# Autodesk Inventor assembly: MX-106T+idle.ipt
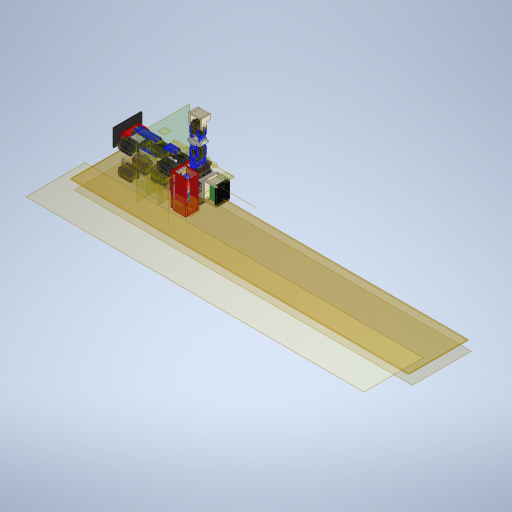
[picture p0: Inventor's stored thumbnail of the model, 512x512]
Saved by Autodesk Inventor 2024 (Build 280153000, 153)
## iProperties
Created: 2022-08-09
Part Number: MX-106T+idle.ipt
Document SubType Name: Assembly
Designer: 박지훈
Author: 박지훈
## Documents named in this file (48)
- C:\Users\Eungang\Documents\Inventor\Fighting_Robot\다이나믹셀\MX-106T+idle.ipt.iam
- C:\Users\Eungang\Documents\Inventor\Fighting_Robot\아이들러\64아이들러.iam
- C:\Users\Eungang\Documents\Inventor\Fighting_Robot\다이나믹셀\MX-106T.ipt
- C:\Users\Eungang\Documents\Inventor\Fighting_Robot\혼\64-106Horn.ipt
- C:\Users\Eungang\Documents\Inventor\Fighting_Robot\new_foot_connect.ipt
- C:\Users\Eungang\Documents\Inventor\Fighting_Robot\foot_2.ipt
- C:\Users\Eungang\Documents\Inventor\Fighting_Robot\new_foot_connect_1.ipt
- C:\Users\Eungang\Documents\Inventor\Fighting_Robot\다이나믹셀\MX-64T.ipt
- C:\Users\Eungang\Documents\Inventor\Fighting_Robot\new_waist.ipt
- C:\Users\Eungang\Documents\Inventor\Fighting_Robot\foot_connect_3_MIR1_MIR1.ipt
- C:\Users\Eungang\Documents\Inventor\Fighting_Robot\real_waist.ipt
- C:\Users\Eungang\Documents\Inventor\Fighting_Robot\Enrichpower_2200mAh_11.1V_30C.ipt
- C:\Users\Eungang\Documents\Inventor\Fighting_Robot\다이나믹셀\MX-28T_R.ipt
- C:\Users\Eungang\Documents\Inventor\Fighting_Robot\혼\28Horn.ipt
- C:\Users\Eungang\Documents\Inventor\Fighting_Robot\아이들러\28아이들러.iam
- C:\Users\Eungang\Documents\Inventor\Fighting_Robot\arm_connect_3.ipt
- C:\Users\Eungang\Documents\Inventor\Fighting_Robot\arm_connect_5.ipt
- C:\Users\Eungang\Documents\Inventor\Fighting_Robot\arm_connect_7.ipt
- C:\Users\Eungang\Documents\Inventor\Fighting_Robot\MOLRA.ipt
- C:\Users\Eungang\Documents\Inventor\Fighting_Robot\a.ipt
- C:\Users\Eungang\Documents\Inventor\Fighting_Robot\Circuit.ipt
- C:\Users\Eungang\Documents\Inventor\Fighting_Robot\neck.ipt
- C:\Users\Eungang\Documents\Inventor\Fighting_Robot\b.ipt
- C:\Users\Eungang\Documents\Inventor\Fighting_Robot\arm_connect_5_MIR.ipt
- C:\Users\Eungang\Documents\Inventor\Fighting_Robot\c.ipt
- C:\Users\Eungang\Documents\Inventor\Fighting_Robot\D.ipt
- C:\Users\Eungang\Documents\Inventor\Fighting_Robot\E.ipt
- C:\Users\Eungang\Documents\Inventor\Fighting_Robot\afdas.ipt
- C:\Users\Eungang\Documents\Inventor\Fighting_Robot\afsd.ipt
- C:\Users\Eungang\Documents\Inventor\Fighting_Robot\afsd_MIR.ipt
- C:\Users\Eungang\Documents\Inventor\Fighting_Robot\adsa.ipt
- C:\Users\Eungang\Documents\Inventor\Fighting_Robot\부품43.ipt
- C:\Users\Eungang\Documents\Inventor\Fighting_Robot\부품44.ipt
- C:\Users\Eungang\Documents\Inventor\Fighting_Robot\64horn.ipt
- C:\Users\Eungang\Documents\Inventor\Fighting_Robot\부품46.ipt
- C:\Users\Eungang\Documents\Inventor\Fighting_Robot\부품47.ipt
- C:\Users\Eungang\Documents\Inventor\Fighting_Robot\부품48.ipt
- C:\Users\Eungang\Documents\Inventor\Fighting_Robot\부품49.ipt
- C:\Users\Eungang\Documents\Inventor\Fighting_Robot\부품50.ipt
- C:\Users\Eungang\Documents\Inventor\Fighting_Robot\부품51.ipt
- C:\Users\Eungang\Documents\Inventor\Fighting_Robot\부품52.ipt
- C:\Users\Eungang\Documents\Inventor\Fighting_Robot\부품53.ipt
- C:\Users\Eungang\Documents\Inventor\Fighting_Robot\부품54.ipt
- C:\Users\Eungang\Documents\Inventor\Fighting_Robot\부품56.ipt
- C:\Users\Eungang\Documents\Inventor\Fighting_Robot\final.ipt
- C:\Users\Eungang\Documents\Inventor\Fighting_Robot\sad.ipt
- C:\Users\Eungang\Documents\Inventor\Fighting_Robot\부품48_MIR.ipt
- C:\Users\Eungang\Documents\Inventor\Fighting_Robot\foot_connect_3_MIR1_MIR1_MIR.ipt
## Components (99 placed, 47 different names)
1. 64-106Horn:1 — 메이트:11, 삽입:35
2. 64-106Horn:2 — 삽입:157, 메이트:405
3. new_foot_connect:2 — 메이트:11, 삽입:180
4. foot_2:1 — 삽입:180, 메이트:402, 플러쉬:100
5. 64-106Horn:5 — 삽입:150, 메이트:404
6. 64아이들러:2 [sub-assembly] — 삽입:165
7. 64아이들러:5 [sub-assembly] — 삽입:164
8. new_foot_connect_1:2
9. MX-64T:3 — 삽입:35, 메이트:325, 플러쉬:77
10. 64아이들러:6 [sub-assembly] — 삽입:189, 플러쉬:88, 메이트:347
11. real_waist:2 — 메이트:218, 플러쉬:78, 메이트:382, 메이트:385, 메이트:396
12. MX-64T:10 — 삽입:100, 삽입:116, 메이트:207, 플러쉬:65, 메이트:360
13. 64-106Horn:12 — 삽입:100, 삽입:185, 삽입:186
14. 64-106Horn:14 — 삽입:117, 메이트:219, 삽입:138
15. arm_connect_7:1
16. a:1 — 메이트:250, 플러쉬:67, 메이트:372, 메이트:374, 메이트:375, 메이트:376
17. 64아이들러:11 [sub-assembly] — 삽입:116
18. neck:1
19. Circuit:1 — 메이트:250, 메이트:370, 메이트:373
20. arm_connect_5:5
21. MX-64T:11 — 플러쉬:65, 메이트:218, 삽입:117, 메이트:219, 플러쉬:66, 메이트:241, 메이트:242, 메이트:337, 플러쉬:79, 메이트:361, 삽입:198, 삽입:199
22. arm_connect_5:6
23. arm_connect_5:7 — 메이트:380, 메이트:381
24. b:1 — 플러쉬:66
25. arm_connect_5:8 — 메이트:377, 메이트:378
26. arm_connect_5_MIR:1
27. MX-28T_R:4 — 메이트:241, 메이트:242, 플러쉬:68, 삽입:132, 삽입:135, 메이트:259
28. c:1 — 플러쉬:67, 메이트:353, 메이트:354, 메이트:355, 메이트:370, 메이트:372, 메이트:373, 메이트:374
29. a:3 — 메이트:353, 메이트:354, 메이트:355
30. D:1 — 플러쉬:68
31. 28Horn:5 — 삽입:132, 삽입:133, 메이트:259
32. arm_connect_3:1 — 삽입:133, 메이트:258
33. 28아이들러:1 [sub-assembly] — 삽입:135, 삽입:136, 삽입:137
34. arm_connect_3:2 — 삽입:136, 삽입:137, 플러쉬:69, 메이트:257
35. E:1 — 플러쉬:69, 메이트:257, 메이트:258, 삽입:138
36. MX-106T:8 — 삽입:150, 삽입:164, 플러쉬:75, 삽입:176, 플러쉬:85, 플러쉬:86, 메이트:345, 삽입:182, 삽입:183, 삽입:184, 메이트:404, 플러쉬:104
37. new_foot_connect_1:3
38. MX-28T_R:5 — 삽입:159, 메이트:289, 메이트:290, 메이트:291, 삽입:201, 메이트:397
39. MX-106T:9 — 삽입:157, 삽입:165, 플러쉬:75, 메이트:325, 플러쉬:77, 메이트:405, 플러쉬:101, 플러쉬:103, 메이트:406, 메이트:407, 메이트:408, 메이트:409
40. 28Horn:6 — 삽입:159, 메이트:289, 메이트:290, 메이트:291, 플러쉬:93, 삽입:200
41. afdas:1
42. foot_connect_3_MIR1_MIR1:2 — 삽입:177
43. afsd_MIR:1 — 삽입:176, 삽입:182
44. new_waist:1 — 삽입:178, 삽입:179, 플러쉬:91, 플러쉬:92, 메이트:356, 메이트:357, 메이트:358, 대칭:2
45. 64아이들러:12 [sub-assembly] — 삽입:177, 삽입:178, 삽입:179
46. adsa:1 — 플러쉬:79
47. 부품43:1
48. MX-106T:10 — 플러쉬:85, 플러쉬:86, 메이트:344, 메이트:345, 삽입:189, 메이트:347, 삽입:190, 플러쉬:89, 메이트:352, 플러쉬:90, 메이트:361, 플러쉬:108
49. 부품44:1
50. afsd:1 — 삽입:183, 삽입:184
51. 64horn:2 — 삽입:185, 삽입:186, 메이트:359
52. 부품47:1 — 플러쉬:88
53. 64-106Horn:17 — 삽입:190, 삽입:191, 삽입:192
54. 부품46:1 — 삽입:191, 삽입:192
55. 64-106Horn:18 — 삽입:194
56. MX-64T:12 — 삽입:194, 플러쉬:89, 메이트:352
57. 부품48:1 — 플러쉬:90
58. 부품49:1 — 메이트:356, 메이트:357, 메이트:358, 메이트:359, 대칭:2
59. MX-64T:14 — 플러쉬:102, 플러쉬:105
60. 부품51:1 — 삽입:198, 삽입:199, 메이트:375, 메이트:376
61. 부품52:1 — 메이트:377, 메이트:378, 메이트:380, 메이트:381
62. 부품50:1 — 메이트:382, 메이트:386, 메이트:387
63. MOLRA:6 — 메이트:391, 메이트:392, 메이트:393
64. 부품50:2 — 메이트:388, 메이트:389, 메이트:390, 메이트:391, 메이트:392, 메이트:393
65. MOLRA:7 — 메이트:385, 메이트:386, 메이트:387, 메이트:388, 메이트:389, 메이트:390
66. Enrichpower_2200mAh_11.1V_30C:1 — 메이트:396
67. 부품53:1 — 플러쉬:93, 삽입:200, 메이트:401
68. 28아이들러:2 [sub-assembly] — 삽입:201, 메이트:397, 플러쉬:95, 삽입:202
69. 부품56:1 — 플러쉬:95, 메이트:398, 메이트:399, 메이트:400, 삽입:202
70. 부품54:1 — 메이트:398, 메이트:399, 메이트:400, 메이트:401
71. final:1 — 메이트:402, 플러쉬:100
72. sad:1 — 플러쉬:101
73. MX-106T:11 — 플러쉬:102, 플러쉬:103, 메이트:406, 플러쉬:106, 삽입:208, 메이트:410, 삽입:212, 삽입:225, 메이트:412, 플러쉬:110, 플러쉬:111, 메이트:415
74. MX-106T:12 — 플러쉬:104, 플러쉬:105, 플러쉬:106, 플러쉬:107, 플러쉬:109, 삽입:205, 삽입:209, 삽입:216, 삽입:217, 삽입:219, 삽입:220
75. new_foot_connect:3 — 삽입:204
76. 64아이들러:13 [sub-assembly] — 삽입:203, 삽입:204
77. 부품48_MIR:1 — 메이트:407, 메이트:408, 메이트:409, 삽입:203
78. MX-106T:13 — 플러쉬:107, 플러쉬:108, 플러쉬:109, 삽입:207, 삽입:210, 삽입:222, 삽입:223
79. 64아이들러:14 [sub-assembly] — 삽입:205, 삽입:214
80. 64아이들러:16 [sub-assembly] — 삽입:207, 삽입:215
81. 64-106Horn:19 — 삽입:208
82. 64-106Horn:20 — 삽입:210, 삽입:221
83. 64-106Horn:21 — 삽입:209, 삽입:211
84. new_foot_connect_1:4 — 삽입:211, 메이트:410
85. new_foot_connect_1:5 — 삽입:213, 삽입:214
86. 64아이들러:17 [sub-assembly] — 삽입:212, 삽입:213
87. 부품47:3 — 삽입:215, 삽입:218
88. afsd_MIR:2 — 삽입:216, 삽입:217, 삽입:218
89. 부품46:2 — 삽입:221, 메이트:411
90. afsd:2 — 삽입:219, 삽입:220, 메이트:411
91. foot_connect_3_MIR1_MIR1_MIR:1 — 삽입:222, 삽입:223, 삽입:224
92. 64아이들러:18 [sub-assembly] — 삽입:224
93. 부품48_MIR:2 — 삽입:225, 메이트:412, 삽입:226
94. new_foot_connect:4 — 삽입:227, 삽입:228, 메이트:413, 메이트:415
95. 64아이들러:19 [sub-assembly] — 삽입:226, 삽입:227
96. foot_2:2 — 삽입:228, 메이트:413, 삽입:229, 삽입:230
97. new_foot_connect:5 — 삽입:229, 삽입:230, 메이트:414
98. MX-64T:15 — 플러쉬:110, 플러쉬:111
99. 64-106Horn:22 — 메이트:414
## Relationships (163: Mate 68, Insert 62, Flush 32, Symmetry 1)
- 플러쉬:1 [Flush] (-30 mm)
- 플러쉬:2 [Flush] (30 mm)
- 메이트:11 [Mate]: 64-106Horn:1 ↔ new_foot_connect:2
- 삽입:35 [Insert] (0.5 mm): 64-106Horn:1 ↔ MX-64T:3
- 삽입:100 [Insert] (0.5 mm): MX-64T:10 ↔ 64-106Horn:12
- 삽입:116 [Insert] (0.5 mm): MX-64T:10 ↔ 64아이들러:11
- 메이트:207 [Mate]: MX-64T:10
- 플러쉬:65 [Flush]: MX-64T:10 ↔ MX-64T:11
- 메이트:218 [Mate]: real_waist:2 ↔ MX-64T:11
- 삽입:117 [Insert] (0.5 mm): 64-106Horn:14 ↔ MX-64T:11
- 메이트:219 [Mate]: 64-106Horn:14 ↔ MX-64T:11
- 플러쉬:66 [Flush]: MX-64T:11 ↔ b:1
- 메이트:241 [Mate]: MX-64T:11 ↔ MX-28T_R:4
- 메이트:242 [Mate]: MX-64T:11 ↔ MX-28T_R:4
- 메이트:250 [Mate] (10 mm): a:1 ↔ Circuit:1
- 플러쉬:67 [Flush]: a:1 ↔ c:1
- 플러쉬:68 [Flush]: MX-28T_R:4 ↔ D:1
- 삽입:132 [Insert] (0.75 mm): MX-28T_R:4 ↔ 28Horn:5
- 삽입:133 [Insert]: 28Horn:5 ↔ arm_connect_3:1
- 삽입:135 [Insert] (0.75 mm): MX-28T_R:4 ↔ 28아이들러:1
- 삽입:136 [Insert]: 28아이들러:1 ↔ arm_connect_3:2
- 삽입:137 [Insert]: 28아이들러:1 ↔ arm_connect_3:2
- 플러쉬:69 [Flush]: arm_connect_3:2 ↔ E:1
- 메이트:257 [Mate]: arm_connect_3:2 ↔ E:1
- 메이트:258 [Mate]: arm_connect_3:1 ↔ E:1
- 메이트:259 [Mate]: MX-28T_R:4 ↔ 28Horn:5
- 삽입:138 [Insert] (0.1 mm): 64-106Horn:14 ↔ E:1
- 삽입:150 [Insert] (0.5 mm): 64-106Horn:5 ↔ MX-106T:8
- 삽입:157 [Insert] (0.5 mm): 64-106Horn:2 ↔ MX-106T:9
- 삽입:159 [Insert] (0.75 mm): MX-28T_R:5 ↔ 28Horn:6
- 메이트:289 [Mate]: MX-28T_R:5 ↔ 28Horn:6
- 메이트:290 [Mate]: MX-28T_R:5 ↔ 28Horn:6
- 메이트:291 [Mate]: MX-28T_R:5 ↔ 28Horn:6
- 삽입:164 [Insert] (0.5 mm): 64아이들러:5 ↔ MX-106T:8
- 삽입:165 [Insert] (0.5 mm): 64아이들러:2 ↔ MX-106T:9
- 플러쉬:75 [Flush]: MX-106T:8 ↔ MX-106T:9
- 삽입:176 [Insert]: MX-106T:8 ↔ afsd_MIR:1
- 메이트:324 [Mate]
- 메이트:325 [Mate]: MX-64T:3 ↔ MX-106T:9
- 플러쉬:77 [Flush]: MX-64T:3 ↔ MX-106T:9
- 삽입:177 [Insert] (0.1 mm): foot_connect_3_MIR1_MIR1:2 ↔ 64아이들러:12
- 삽입:178 [Insert]: new_waist:1 ↔ 64아이들러:12
- 삽입:179 [Insert]: new_waist:1 ↔ 64아이들러:12
- 플러쉬:78 [Flush] (-6 mm): real_waist:2
- 메이트:337 [Mate]: MX-64T:11
- 플러쉬:79 [Flush]: MX-64T:11 ↔ adsa:1
- 삽입:180 [Insert]: new_foot_connect:2 ↔ foot_2:1
- 플러쉬:85 [Flush]: MX-106T:8 ↔ MX-106T:10
- 플러쉬:86 [Flush]: MX-106T:8 ↔ MX-106T:10
- 메이트:344 [Mate]: MX-106T:10
- 메이트:345 [Mate] (20 mm): MX-106T:8 ↔ MX-106T:10
- 삽입:182 [Insert]: MX-106T:8 ↔ afsd_MIR:1
- 삽입:183 [Insert]: MX-106T:8 ↔ afsd:1
- 삽입:184 [Insert]: MX-106T:8 ↔ afsd:1
- 삽입:185 [Insert]: 64-106Horn:12 ↔ 64horn:2
- 삽입:186 [Insert]: 64-106Horn:12 ↔ 64horn:2
- 삽입:189 [Insert] (0.5 mm): 64아이들러:6 ↔ MX-106T:10
- 플러쉬:88 [Flush]: 64아이들러:6 ↔ 부품47:1
- 메이트:347 [Mate]: 64아이들러:6 ↔ MX-106T:10
- 삽입:190 [Insert] (0.5 mm): MX-106T:10 ↔ 64-106Horn:17
- 삽입:191 [Insert]: 64-106Horn:17 ↔ 부품46:1
- 삽입:192 [Insert]: 64-106Horn:17 ↔ 부품46:1
- 삽입:194 [Insert] (0.5 mm): 64-106Horn:18 ↔ MX-64T:12
- 플러쉬:89 [Flush]: MX-106T:10 ↔ MX-64T:12
- 메이트:352 [Mate]: MX-106T:10 ↔ MX-64T:12
- 플러쉬:90 [Flush]: MX-106T:10 ↔ 부품48:1
- 메이트:353 [Mate]: c:1 ↔ a:3
- 메이트:354 [Mate]: c:1 ↔ a:3
- 메이트:355 [Mate]: c:1 ↔ a:3
- 플러쉬:91 [Flush]: new_waist:1
- 플러쉬:92 [Flush]: new_waist:1
- 메이트:356 [Mate]: new_waist:1 ↔ 부품49:1
- 메이트:357 [Mate]: new_waist:1 ↔ 부품49:1
- 메이트:358 [Mate]: new_waist:1 ↔ 부품49:1
- 메이트:359 [Mate]: 64horn:2 ↔ 부품49:1
- 대칭:2 [Symmetry]: new_waist:1 ↔ 부품49:1
- 메이트:360 [Mate]: MX-64T:10
- 메이트:361 [Mate]: MX-64T:11 ↔ MX-106T:10
- 메이트:370 [Mate] (0.2 mm): Circuit:1 ↔ c:1
- 메이트:372 [Mate]: a:1 ↔ c:1
- 메이트:373 [Mate] (0.2 mm): Circuit:1 ↔ c:1
- 삽입:198 [Insert]: MX-64T:11 ↔ 부품51:1
- 삽입:199 [Insert]: MX-64T:11 ↔ 부품51:1
- 메이트:374 [Mate]: a:1 ↔ c:1
- 메이트:375 [Mate]: a:1 ↔ 부품51:1
- 메이트:376 [Mate]: a:1 ↔ 부품51:1
- 메이트:377 [Mate] (0.1 mm): arm_connect_5:8 ↔ 부품52:1
- 메이트:378 [Mate]: arm_connect_5:8 ↔ 부품52:1
- 메이트:380 [Mate]: arm_connect_5:7 ↔ 부품52:1
- 메이트:381 [Mate]: arm_connect_5:7 ↔ 부품52:1
- 메이트:382 [Mate]: real_waist:2 ↔ 부품50:1
- 메이트:385 [Mate]: real_waist:2 ↔ MOLRA:7
- 메이트:386 [Mate]: 부품50:1 ↔ MOLRA:7
- 메이트:387 [Mate]: 부품50:1 ↔ MOLRA:7
- 메이트:388 [Mate]: 부품50:2 ↔ MOLRA:7
- 메이트:389 [Mate]: 부품50:2 ↔ MOLRA:7
- 메이트:390 [Mate]: 부품50:2 ↔ MOLRA:7
- 메이트:391 [Mate]: MOLRA:6 ↔ 부품50:2
- 메이트:392 [Mate]: MOLRA:6 ↔ 부품50:2
- 메이트:393 [Mate]: MOLRA:6 ↔ 부품50:2
- 메이트:396 [Mate]: real_waist:2 ↔ Enrichpower_2200mAh_11.1V_30C:1
- 플러쉬:93 [Flush]: 28Horn:6 ↔ 부품53:1
- 삽입:200 [Insert]: 28Horn:6 ↔ 부품53:1
- 삽입:201 [Insert] (0.5 mm): MX-28T_R:5 ↔ 28아이들러:2
- 메이트:397 [Mate]: MX-28T_R:5 ↔ 28아이들러:2
- 플러쉬:95 [Flush]: 28아이들러:2 ↔ 부품56:1
- 메이트:398 [Mate]: 부품56:1 ↔ 부품54:1
- 메이트:399 [Mate]: 부품56:1 ↔ 부품54:1
- 메이트:400 [Mate]: 부품56:1 ↔ 부품54:1
- 메이트:401 [Mate]: 부품53:1 ↔ 부품54:1
- 메이트:402 [Mate]: foot_2:1 ↔ final:1
- 플러쉬:100 [Flush] (-33 mm): foot_2:1 ↔ final:1
- 메이트:404 [Mate]: 64-106Horn:5 ↔ MX-106T:8
- 메이트:405 [Mate]: 64-106Horn:2 ↔ MX-106T:9
- 삽입:202 [Insert]: 28아이들러:2 ↔ 부품56:1
- 플러쉬:101 [Flush]: MX-106T:9 ↔ sad:1
- 플러쉬:102 [Flush]: MX-64T:14 ↔ MX-106T:11
- 플러쉬:103 [Flush]: MX-106T:9 ↔ MX-106T:11
- 메이트:406 [Mate]: MX-106T:9 ↔ MX-106T:11
- 플러쉬:104 [Flush]: MX-106T:8 ↔ MX-106T:12
- 플러쉬:105 [Flush]: MX-64T:14 ↔ MX-106T:12
- 플러쉬:106 [Flush]: MX-106T:11 ↔ MX-106T:12
- 메이트:407 [Mate]: MX-106T:9 ↔ 부품48_MIR:1
- 메이트:408 [Mate]: MX-106T:9 ↔ 부품48_MIR:1
- 메이트:409 [Mate]: MX-106T:9 ↔ 부품48_MIR:1
- 삽입:203 [Insert]: 64아이들러:13 ↔ 부품48_MIR:1
- 삽입:204 [Insert]: new_foot_connect:3 ↔ 64아이들러:13
- 플러쉬:107 [Flush]: MX-106T:12 ↔ MX-106T:13
- 플러쉬:108 [Flush]: MX-106T:10 ↔ MX-106T:13
- 플러쉬:109 [Flush]: MX-106T:12 ↔ MX-106T:13
- 삽입:205 [Insert] (0.5 mm): MX-106T:12 ↔ 64아이들러:14
- 삽입:207 [Insert] (0.5 mm): MX-106T:13 ↔ 64아이들러:16
- 삽입:208 [Insert] (0.5 mm): MX-106T:11 ↔ 64-106Horn:19
- 삽입:209 [Insert] (0.5 mm): MX-106T:12 ↔ 64-106Horn:21
- 삽입:210 [Insert] (0.5 mm): MX-106T:13 ↔ 64-106Horn:20
- 삽입:211 [Insert]: 64-106Horn:21 ↔ new_foot_connect_1:4
- 메이트:410 [Mate]: MX-106T:11 ↔ new_foot_connect_1:4
- 삽입:212 [Insert] (0.5 mm): MX-106T:11 ↔ 64아이들러:17
- 삽입:213 [Insert]: new_foot_connect_1:5 ↔ 64아이들러:17
- 삽입:214 [Insert]: 64아이들러:14 ↔ new_foot_connect_1:5
- 삽입:215 [Insert]: 64아이들러:16 ↔ 부품47:3
- 삽입:216 [Insert]: MX-106T:12 ↔ afsd_MIR:2
- 삽입:217 [Insert]: MX-106T:12 ↔ afsd_MIR:2
- 삽입:218 [Insert] (0.2 mm): 부품47:3 ↔ afsd_MIR:2
- 삽입:219 [Insert]: MX-106T:12 ↔ afsd:2
- 삽입:220 [Insert]: MX-106T:12 ↔ afsd:2
- 삽입:221 [Insert]: 64-106Horn:20 ↔ 부품46:2
- 메이트:411 [Mate] (0.2 mm): 부품46:2 ↔ afsd:2
- 삽입:222 [Insert]: MX-106T:13 ↔ foot_connect_3_MIR1_MIR1_MIR:1
- 삽입:223 [Insert]: MX-106T:13 ↔ foot_connect_3_MIR1_MIR1_MIR:1
- 삽입:224 [Insert]: foot_connect_3_MIR1_MIR1_MIR:1 ↔ 64아이들러:18
- 삽입:225 [Insert]: MX-106T:11 ↔ 부품48_MIR:2
- 메이트:412 [Mate]: MX-106T:11 ↔ 부품48_MIR:2
- 삽입:226 [Insert]: 부품48_MIR:2 ↔ 64아이들러:19
- 삽입:227 [Insert]: new_foot_connect:4 ↔ 64아이들러:19
- 삽입:228 [Insert]: new_foot_connect:4 ↔ foot_2:2
- 메이트:413 [Mate]: new_foot_connect:4 ↔ foot_2:2
- 삽입:229 [Insert]: foot_2:2 ↔ new_foot_connect:5
- 삽입:230 [Insert]: foot_2:2 ↔ new_foot_connect:5
- 플러쉬:110 [Flush]: MX-106T:11 ↔ MX-64T:15
- 플러쉬:111 [Flush]: MX-106T:11 ↔ MX-64T:15
- 메이트:414 [Mate]: new_foot_connect:5 ↔ 64-106Horn:22
- 메이트:415 [Mate]: MX-106T:11 ↔ new_foot_connect:4
